# Autodesk Inventor assembly: Assembly1iiiiii
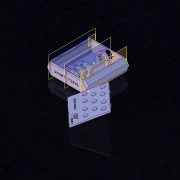
[picture p0: Inventor's stored thumbnail of the model, 180x180]
Saved by Autodesk Inventor 2016 (Build 200138000, 138)
## iProperties
Created: 2018-01-03
Part Number: Assembly1iiiiii
Document SubType Name: Assembly
Designer: ALIREZA
Author: ALIREZA
## Documents named in this file (5)
- C:\Users\ALIREZA\Desktop\Cad files inventor\Assembly1iiiiii.iam
- C:\Users\ALIREZA\Desktop\Cad files inventor\Frame2.ipt
- C:\Users\ALIREZA\Desktop\Cad files inventor\Frame2CAP2.ipt
- C:\Users\ALIREZA\Desktop\Cad files inventor\ROTATION2.ipt
- C:\Users\ALIREZA\Desktop\Cad files inventor\motor holder.ipt
## Components (6 placed, 4 different names)
1. Frame2:1 — Mate:1, Mate:3, Mate:4, Mate:5
2. Frame2CAP2:1
3. ROTATION2:1 — Mate:1
4. motor holder:1 — Mate:4
5. motor holder:2 — Mate:3
6. motor holder:3 — Mate:5
## Relationships (4: Mate 4)
- Mate:1: Frame2:1 ↔ ROTATION2:1
- Mate:3: Frame2:1 ↔ motor holder:2
- Mate:4: Frame2:1 ↔ motor holder:1
- Mate:5: Frame2:1 ↔ motor holder:3
